# Autodesk Inventor assembly: claw_nut_test
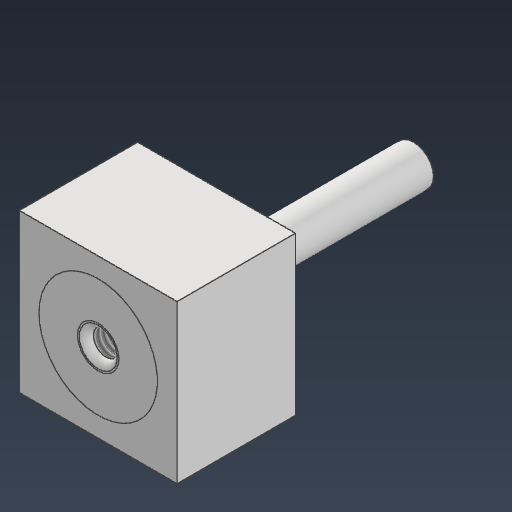
[picture p0: Inventor's stored thumbnail of the model, 512x512]
Saved by Autodesk Inventor 2023 (Build 270158000, 158)
## iProperties
Created: 2026-01-23
Part Number: claw_nut_test
Document SubType Name: Assembly
Designer: szymo
Author: szymo
## Documents named in this file (3)
- D:\tech\diy\e-skateboard\projekcik-inventor\claw_nut_test.iam
- D:\tech\diy\e-skateboard\projekcik-inventor\claw_nut_test.ipt
- D:\tech\diy\e-skateboard\projekcik-inventor\claw_nut.ipt
## Components (2 placed, 2 different names)
1. claw_nut_test:1 — Mate:1, Flush:1
2. claw_nut:1 — Mate:1, Flush:1
## Relationships (2: Mate 1, Flush 1)
- Mate:1: claw_nut_test:1 ↔ claw_nut:1
- Flush:1: claw_nut_test:1 ↔ claw_nut:1
